# Autodesk Inventor assembly: sideassembly(sa)_MIR
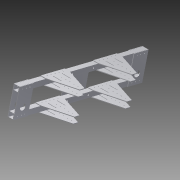
[picture p0: Inventor's stored thumbnail of the model, 180x180]
Saved by Autodesk Inventor 2015 (Build 190159000, 159)
## iProperties
Created: 2015-10-03
Part Number: sideassembly(sa)_MIR
Document SubType Name: Assembly
Designer: elilitwack
Mass: 2214.44 g
Surface Area: 7372.09 cm^2
Volume: 820.163 cm^3
Density: 2.7 g/cm^3
Author: elilitwack
## Documents named in this file (6)
- C:\Users\elilitwack\Documents\2015 Offseason Chassis\West Coast Chassis Fall 2015 - iLogic\sideassembly(sa)_MIR.iam
- C:\Users\elilitwack\Documents\2015 Offseason Chassis\West Coast Chassis Fall 2015 - iLogic\sidetube(st_MIR.ipt
- C:\Users\elilitwack\Documents\2015 Offseason Chassis\West Coast Chassis Fall 2015 - iLogic\bearingplate(bp)_MIR.ipt
- C:\Users\elilitwack\Documents\2015 Offseason Chassis\West Coast Chassis Fall 2015 - iLogic\gearboxbearingplate(gbpb)_MIR.ipt
- C:\Users\elilitwack\Documents\2015 Offseason Chassis\West Coast Chassis Fall 2015 - iLogic\traingle_bracket(tb)_MIR.ipt
- C:\Users\elilitwack\Documents\2015 Offseason Chassis\West Coast Chassis Fall 2015 - iLogic\traingle_bracket(tb).ipt
## Components (15 placed, 5 different names)
1. sidetube(st_MIR:1 — Mate:14, Mate:12, Mate:11, Mate:13, Mate:10, Mate:9, Mate:29, Mate:28, Mate:27, Mate:38, Mate:37, Mate:36, Mate:35, Mate:34, Mate:33, Mate:59, Mate:58, Mate:57, Mate:62, Mate:61, Mate:60, Mate:50, Mate:49, Mate:48, Mate:63, Mate:64, Mate:65
2. sidetube(st_MIR:2 — Mate:19, Mate:18, Mate:17, Mate:20, Mate:16, Mate:15, Mate:53, Mate:52, Mate:51, Mate:56, Mate:55, Mate:54, Mate:65, Mate:64, Mate:63, Mate:68, Mate:67, Mate:66
3. bearingplate(bp)_MIR:1 — Mate:19, Mate:18, Mate:17, Mate:14, Mate:12, Mate:11
4. bearingplate(bp)_MIR:2 — Mate:20, Mate:16, Mate:15, Mate:13, Mate:10, Mate:9
5. gearboxbearingplate(gbpb)_MIR:1 — Mate:29, Mate:28, Mate:27
6. bearingplate(bp)_MIR:3 — Mate:38, Mate:37, Mate:36
7. bearingplate(bp)_MIR:4 — Mate:35, Mate:34, Mate:33
8. traingle_bracket(tb)_MIR:2 — Mate:59, Mate:58, Mate:57
9. traingle_bracket(tb)_MIR:3 — Mate:62, Mate:61, Mate:60
10. traingle_bracket(tb)_MIR:4 — Mate:50, Mate:49, Mate:48
11. traingle_bracket(tb)_MIR:5 — Mate:53, Mate:52, Mate:51
12. traingle_bracket(tb)_MIR:6 — Mate:56, Mate:55, Mate:54
13. traingle_bracket(tb)_MIR:7 — Mate:65, Mate:64, Mate:63
14. traingle_bracket(tb)_MIR:8 — Mate:68, Mate:67, Mate:66
15. traingle_bracket(tb):1 — Mate:63, Mate:64, Mate:65
## Relationships (45: Mate 45)
- Mate:19: sidetube(st_MIR:2 ↔ bearingplate(bp)_MIR:1
- Mate:18: sidetube(st_MIR:2 ↔ bearingplate(bp)_MIR:1
- Mate:17: sidetube(st_MIR:2 ↔ bearingplate(bp)_MIR:1
- Mate:14: sidetube(st_MIR:1 ↔ bearingplate(bp)_MIR:1
- Mate:12: sidetube(st_MIR:1 ↔ bearingplate(bp)_MIR:1
- Mate:11: sidetube(st_MIR:1 ↔ bearingplate(bp)_MIR:1
- Mate:20: sidetube(st_MIR:2 ↔ bearingplate(bp)_MIR:2
- Mate:16: sidetube(st_MIR:2 ↔ bearingplate(bp)_MIR:2
- Mate:15: sidetube(st_MIR:2 ↔ bearingplate(bp)_MIR:2
- Mate:13: sidetube(st_MIR:1 ↔ bearingplate(bp)_MIR:2
- Mate:10: sidetube(st_MIR:1 ↔ bearingplate(bp)_MIR:2
- Mate:9: sidetube(st_MIR:1 ↔ bearingplate(bp)_MIR:2
- Mate:29: sidetube(st_MIR:1 ↔ gearboxbearingplate(gbpb)_MIR:1
- Mate:28: sidetube(st_MIR:1 ↔ gearboxbearingplate(gbpb)_MIR:1
- Mate:27: sidetube(st_MIR:1 ↔ gearboxbearingplate(gbpb)_MIR:1
- Mate:38: sidetube(st_MIR:1 ↔ bearingplate(bp)_MIR:3
- Mate:37: sidetube(st_MIR:1 ↔ bearingplate(bp)_MIR:3
- Mate:36: sidetube(st_MIR:1 ↔ bearingplate(bp)_MIR:3
- Mate:35: sidetube(st_MIR:1 ↔ bearingplate(bp)_MIR:4
- Mate:34: sidetube(st_MIR:1 ↔ bearingplate(bp)_MIR:4
- Mate:33: sidetube(st_MIR:1 ↔ bearingplate(bp)_MIR:4
- Mate:59: sidetube(st_MIR:1 ↔ traingle_bracket(tb)_MIR:2
- Mate:58: sidetube(st_MIR:1 ↔ traingle_bracket(tb)_MIR:2
- Mate:57: sidetube(st_MIR:1 ↔ traingle_bracket(tb)_MIR:2
- Mate:62: sidetube(st_MIR:1 ↔ traingle_bracket(tb)_MIR:3
- Mate:61: sidetube(st_MIR:1 ↔ traingle_bracket(tb)_MIR:3
- Mate:60: sidetube(st_MIR:1 ↔ traingle_bracket(tb)_MIR:3
- Mate:50: sidetube(st_MIR:1 ↔ traingle_bracket(tb)_MIR:4
- Mate:49: sidetube(st_MIR:1 ↔ traingle_bracket(tb)_MIR:4
- Mate:48: sidetube(st_MIR:1 ↔ traingle_bracket(tb)_MIR:4
- Mate:53: sidetube(st_MIR:2 ↔ traingle_bracket(tb)_MIR:5
- Mate:52: sidetube(st_MIR:2 ↔ traingle_bracket(tb)_MIR:5
- Mate:51: sidetube(st_MIR:2 ↔ traingle_bracket(tb)_MIR:5
- Mate:56: sidetube(st_MIR:2 ↔ traingle_bracket(tb)_MIR:6
- Mate:55: sidetube(st_MIR:2 ↔ traingle_bracket(tb)_MIR:6
- Mate:54: sidetube(st_MIR:2 ↔ traingle_bracket(tb)_MIR:6
- Mate:65: sidetube(st_MIR:2 ↔ traingle_bracket(tb)_MIR:7
- Mate:64: sidetube(st_MIR:2 ↔ traingle_bracket(tb)_MIR:7
- Mate:63: sidetube(st_MIR:2 ↔ traingle_bracket(tb)_MIR:7
- Mate:68: sidetube(st_MIR:2 ↔ traingle_bracket(tb)_MIR:8
- Mate:67: sidetube(st_MIR:2 ↔ traingle_bracket(tb)_MIR:8
- Mate:66: sidetube(st_MIR:2 ↔ traingle_bracket(tb)_MIR:8
- Mate:63: sidetube(st_MIR:1 ↔ traingle_bracket(tb):1
- Mate:64: sidetube(st_MIR:1 ↔ traingle_bracket(tb):1
- Mate:65: sidetube(st_MIR:1 ↔ traingle_bracket(tb):1
